# Autodesk Inventor assembly: torchArm
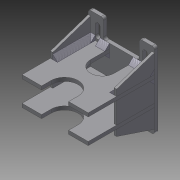
[picture p0: Inventor's stored thumbnail of the model, 180x180]
Saved by Autodesk Inventor 2013 (Build 170138000, 138)
## iProperties
Created: 2012-12-11
Part Number: torchArm
Document SubType Name: Weldment
Designer: istvan.burbank
Weld Material: Aluminum 6061, Welded
Author: istvan.burbank
## Documents named in this file (5)
- E:\GitHub\Crown-Fire\CAD\CuttingHead\torchArm.iam
- E:\GitHub\Crown-Fire\CAD\CuttingHead\torchArm.ipt
- E:\GitHub\Crown-Fire\CAD\CuttingHead\triangleBrace.ipt
- E:\GitHub\Crown-Fire\CAD\CuttingHead\torchMount_back.ipt
- E:\GitHub\Crown-Fire\CAD\CuttingHead\squareBrace.ipt
## Components (9 placed, 4 different names)
1. torchMount_back:1 — Mate:1, Flush:1, Mate:6, Mate:7, Mate:8, Mate:9, Flush:6, Mate:10, Flush:7, Flush:8, Flush:9, Flush:10, Mate:15, Mate:16
2. torchArm:1 — Mate:1, Flush:1, Mate:2, Mate:3, Flush:2, Flush:3, Flush:4, Flush:5, Flush:6
3. torchArm:3 — Mate:10, Flush:7, Mate:11, Mate:12, Flush:8, Mate:13, Mate:14
4. triangleBrace:1 — Mate:3, Flush:5, Mate:6
5. triangleBrace:2 — Mate:2, Flush:3, Mate:9
6. triangleBrace:3 — Flush:2, Mate:8, Mate:12
7. triangleBrace:4 — Flush:4, Mate:7, Mate:11
8. squareBrace:1 — Flush:10, Mate:13, Mate:15
9. squareBrace:2 — Flush:9, Mate:14, Mate:16
## Relationships (24: Mate 14, Flush 10)
- Mate:1: torchMount_back:1 ↔ torchArm:1
- Flush:1: torchMount_back:1 ↔ torchArm:1
- Mate:2: torchArm:1 ↔ triangleBrace:2
- Mate:3: torchArm:1 ↔ triangleBrace:1
- Flush:2: torchArm:1 ↔ triangleBrace:3
- Flush:3: torchArm:1 ↔ triangleBrace:2
- Flush:4: torchArm:1 ↔ triangleBrace:4
- Flush:5: torchArm:1 ↔ triangleBrace:1
- Mate:6: torchMount_back:1 ↔ triangleBrace:1
- Mate:7: torchMount_back:1 ↔ triangleBrace:4
- Mate:8: torchMount_back:1 ↔ triangleBrace:3
- Mate:9: torchMount_back:1 ↔ triangleBrace:2
- Flush:6 (6.35 mm): torchMount_back:1 ↔ torchArm:1
- Mate:10: torchMount_back:1 ↔ torchArm:3
- Flush:7: torchMount_back:1 ↔ torchArm:3
- Mate:11: torchArm:3 ↔ triangleBrace:4
- Mate:12: torchArm:3 ↔ triangleBrace:3
- Flush:8 (6.35 mm): torchMount_back:1 ↔ torchArm:3
- Flush:9: torchMount_back:1 ↔ squareBrace:2
- Flush:10: torchMount_back:1 ↔ squareBrace:1
- Mate:13: torchArm:3 ↔ squareBrace:1
- Mate:14: torchArm:3 ↔ squareBrace:2
- Mate:15: torchMount_back:1 ↔ squareBrace:1
- Mate:16: torchMount_back:1 ↔ squareBrace:2
